# Autodesk Inventor assembly: TATTU 1300mah 3s
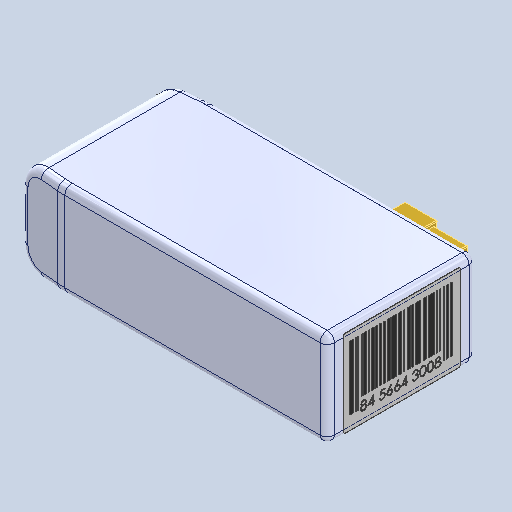
[picture p0: Inventor's stored thumbnail of the model, 512x512]
Saved by Autodesk Inventor 2022.1 (Build 261234020, 234B)
## iProperties
Created: 2016-11-21
Part Number: TATTU 1300mah 3s
Document SubType Name: Assembly
Designer: NCai2
Sending System: SolidWorks 2018
Last Author: Simone
Last Saved: 2018-08-25
Author: NCai2
## Documents named in this file (5)
- D:\Inventor\0.3rd Lawette - V3.0\Tattu 4S 650mah\TATTU 1300mah 3s.iam
- D:\Inventor\0.3rd Lawette - V3.0\Tattu 4S 650mah\FUNDA 13.ipt
- D:\Inventor\0.3rd Lawette - V3.0\Tattu 4S 650mah\tattu 1300MHa 3s LiPo.ipt
- D:\Inventor\0.3rd Lawette - V3.0\Tattu 4S 650mah\JST XHP-4.ipt
- D:\Inventor\0.3rd Lawette - V3.0\Tattu 4S 650mah\XT60 Buchse.ipt
## Components (4 placed, 4 different names)
1. FUNDA 13:1
2. tattu 1300MHa 3s LiPo:1 — Mate:1, Flush:1, Flush:2, Mate:2, Flush:3
3. JST XHP-4:1 — Mate:2, Flush:3, Flush:4
4. XT60 Buchse:2 — Mate:1, Flush:1, Flush:2, Flush:4
## Relationships (6: Flush 4, Mate 2)
- Mate:1: tattu 1300MHa 3s LiPo:1 ↔ XT60 Buchse:2
- Flush:1: tattu 1300MHa 3s LiPo:1 ↔ XT60 Buchse:2
- Flush:2: tattu 1300MHa 3s LiPo:1 ↔ XT60 Buchse:2
- Mate:2: tattu 1300MHa 3s LiPo:1 ↔ JST XHP-4:1
- Flush:3: tattu 1300MHa 3s LiPo:1 ↔ JST XHP-4:1
- Flush:4: JST XHP-4:1 ↔ XT60 Buchse:2
